# Autodesk Inventor assembly: Montagem1
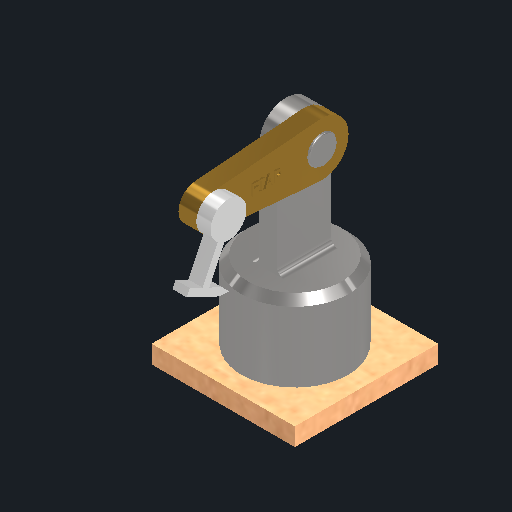
[picture p0: Inventor's stored thumbnail of the model, 512x512]
Saved by Autodesk Inventor 2027 (Build 310192060, 192F)
## iProperties
Created: 2026-08-31
Part Number: Montagem1
Document SubType Name: Assembly
Designer: guisg
Author: guisg
## Documents named in this file (5)
- C:\Users\guisg\Downloads\CP1_CAD\Montagem1.iam
- C:\Users\guisg\Downloads\Peça1.ipt
- C:\Users\guisg\Downloads\peça2.ipt
- C:\Users\guisg\Downloads\Peça3.ipt
- C:\Users\guisg\Downloads\Peça4.ipt
## Components (4 placed, 4 different names)
1. Peça1:1 — Inserir:2, Inserir:3
2. peça2:1 — Inserir:1
3. Peça3:1 — Inserir:1, Inserir:2
4. Peça4:1 — Inserir:3
## Relationships (3: Insert 3)
- Inserir:1: peça2:1 ↔ Peça3:1
- Inserir:2: Peça1:1 ↔ Peça3:1
- Inserir:3 (-2.5 mm): Peça1:1 ↔ Peça4:1
